# Autodesk Inventor assembly: Power Board w. Drivers
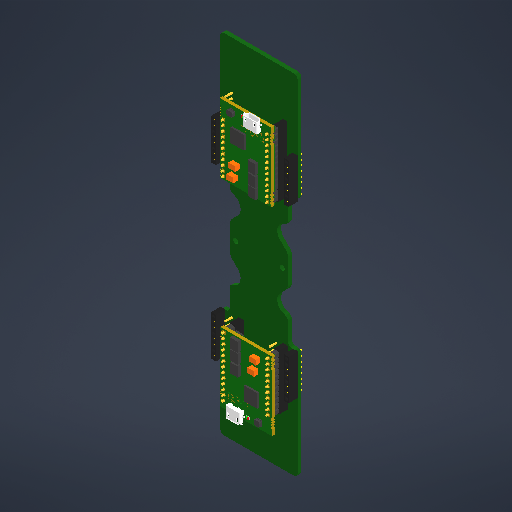
[picture p0: Inventor's stored thumbnail of the model, 512x512]
Saved by Autodesk Inventor 2026.1 (Build 301233020, 233B)
## iProperties
Created: 2025-11-16
Part Number: Power Board w. Drivers
Document SubType Name: Assembly
Designer: Bahaa
Author: Bahaa
## Documents named in this file (6)
- C:\Users\Bahaa\Nextcloud2\CAD\25-26\Boards\Power Board w. Drivers.iam
- C:\Users\Bahaa\Nextcloud2\CAD\25-26\Boards\Power Board.ipt
- C:\Users\Bahaa\Nextcloud2\CAD\25-26\Electronics\466023_escon_module_24-2.ipt
- C:\Users\Bahaa\Nextcloud2\CAD\25-26\Electronics\13-Pin Header - Female - 2.54mm.ipt
- C:\Users\Bahaa\Nextcloud2\CAD\25-26\Electronics\11-Pin Header - Female - 2.54mm.iam
- C:\Users\Bahaa\Nextcloud2\CAD\25-26\Electronics\8-Pin Header - Female - 2.54mm.iam
## Components (13 placed, 5 different names)
1. Power Board:1 — Flush:4, Mate:5, Mate:6, Flush:7, Mate:10, Mate:11, Mate:12, Mate:13, Flush:14, Flush:16, Flush:18, Flush:20, Flush:22, Flush:23, Flush:25, Flush:26, Flush:27, Flush:28, Flush:29, Mate:14, Flush:30, Flush:31, Flush:32, Mate:15
2. 466023_escon_module_24-2:1 — Flush:1, Mate:2, Mate:3, Mate:4, Flush:2, Flush:3, Flush:27
3. 13-Pin Header - Female - 2.54mm:1 — Flush:1, Mate:2, Mate:3, Flush:4, Mate:5
4. 11-Pin Header - Female - 2.54mm:1 [sub-assembly] — Mate:4, Flush:2, Flush:3
5. 466023_escon_module_24-2:2 — Mate:6, Flush:7, Flush:26
6. 466023_escon_module_24-2:3 — Flush:9, Mate:7, Flush:10, Mate:8, Flush:11, Mate:9, Flush:29
7. 466023_escon_module_24-2:4 — Flush:31, Flush:32, Mate:15
8. 13-Pin Header - Female - 2.54mm:2 — Mate:8, Flush:11, Mate:9
9. 11-Pin Header - Female - 2.54mm:2 [sub-assembly] — Flush:9, Mate:7, Flush:10, Mate:14, Flush:30
10. 8-Pin Header - Female - 2.54mm:1 [sub-assembly] — Mate:11, Flush:16, Flush:22
11. 8-Pin Header - Female - 2.54mm:2 [sub-assembly] — Mate:10, Flush:20, Flush:28
12. 8-Pin Header - Female - 2.54mm:3 [sub-assembly] — Mate:12, Flush:14, Flush:23
13. 8-Pin Header - Female - 2.54mm:4 [sub-assembly] — Mate:13, Flush:18, Flush:25
## Relationships (36: Flush 22, Mate 14)
- Flush:1: 466023_escon_module_24-2:1 ↔ 13-Pin Header - Female - 2.54mm:1
- Mate:2: 466023_escon_module_24-2:1 ↔ 13-Pin Header - Female - 2.54mm:1
- Mate:3: 466023_escon_module_24-2:1 ↔ 13-Pin Header - Female - 2.54mm:1
- Mate:4: 466023_escon_module_24-2:1 ↔ 11-Pin Header - Female - 2.54mm:1
- Flush:2: 466023_escon_module_24-2:1 ↔ 11-Pin Header - Female - 2.54mm:1
- Flush:3: 466023_escon_module_24-2:1 ↔ 11-Pin Header - Female - 2.54mm:1
- Flush:4: Power Board:1 ↔ 13-Pin Header - Female - 2.54mm:1
- Mate:5: Power Board:1 ↔ 13-Pin Header - Female - 2.54mm:1
- Mate:6: Power Board:1 ↔ 466023_escon_module_24-2:2
- Flush:7: Power Board:1 ↔ 466023_escon_module_24-2:2
- Flush:9: 466023_escon_module_24-2:3 ↔ 11-Pin Header - Female - 2.54mm:2
- Mate:7: 466023_escon_module_24-2:3 ↔ 11-Pin Header - Female - 2.54mm:2
- Flush:10: 466023_escon_module_24-2:3 ↔ 11-Pin Header - Female - 2.54mm:2
- Mate:8: 466023_escon_module_24-2:3 ↔ 13-Pin Header - Female - 2.54mm:2
- Flush:11: 466023_escon_module_24-2:3 ↔ 13-Pin Header - Female - 2.54mm:2
- Mate:9: 466023_escon_module_24-2:3 ↔ 13-Pin Header - Female - 2.54mm:2
- Mate:10: Power Board:1 ↔ 8-Pin Header - Female - 2.54mm:2
- Mate:11: Power Board:1 ↔ 8-Pin Header - Female - 2.54mm:1
- Mate:12: Power Board:1 ↔ 8-Pin Header - Female - 2.54mm:3
- Mate:13: Power Board:1 ↔ 8-Pin Header - Female - 2.54mm:4
- Flush:14: Power Board:1 ↔ 8-Pin Header - Female - 2.54mm:3
- Flush:16: Power Board:1 ↔ 8-Pin Header - Female - 2.54mm:1
- Flush:18: Power Board:1 ↔ 8-Pin Header - Female - 2.54mm:4
- Flush:20: Power Board:1 ↔ 8-Pin Header - Female - 2.54mm:2
- Flush:22: Power Board:1 ↔ 8-Pin Header - Female - 2.54mm:1
- Flush:23: Power Board:1 ↔ 8-Pin Header - Female - 2.54mm:3
- Flush:25: Power Board:1 ↔ 8-Pin Header - Female - 2.54mm:4
- Flush:26: Power Board:1 ↔ 466023_escon_module_24-2:2
- Flush:27: Power Board:1 ↔ 466023_escon_module_24-2:1
- Flush:28: Power Board:1 ↔ 8-Pin Header - Female - 2.54mm:2
- Flush:29: Power Board:1 ↔ 466023_escon_module_24-2:3
- Mate:14: Power Board:1 ↔ 11-Pin Header - Female - 2.54mm:2
- Flush:30: Power Board:1 ↔ 11-Pin Header - Female - 2.54mm:2
- Flush:31: Power Board:1 ↔ 466023_escon_module_24-2:4
- Flush:32: Power Board:1 ↔ 466023_escon_module_24-2:4
- Mate:15: Power Board:1 ↔ 466023_escon_module_24-2:4
